# Autodesk Inventor assembly: ASY GBK 1320 long wall shield 5
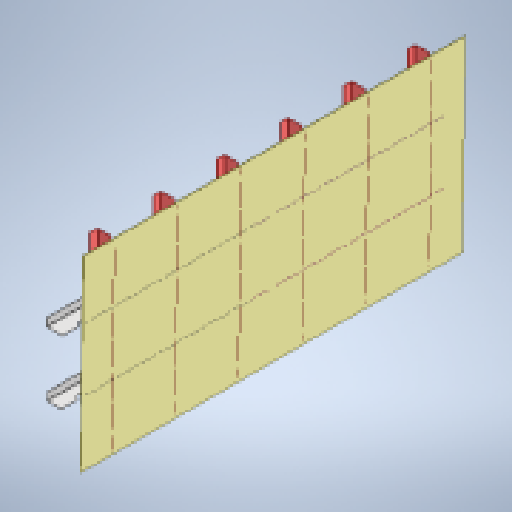
[picture p0: Inventor's stored thumbnail of the model, 512x512]
Saved by Autodesk Inventor 2026 (Build 300175000, 175)
## iProperties
Created: 2026-05-07
Part Number: ASY GBK 1320 long wall shield 5
Document SubType Name: Assembly
Designer: pokla
Mass: 215512 g
Surface Area: 139105 cm^2
Volume: 27453.8 cm^3
Density: 7.85 g/cm^3
Stock Number: 1321
Author: admin
## Documents named in this file (6)
- C:\Users\pokla\Documents\Inventor\GBK-Gubkinskiy\ASY GBK 1320 long wall shield 5.iam
- C:\Users\pokla\Documents\Inventor\GBK-Gubkinskiy\GBK 1211 shield 2.ipt
- C:\Users\pokla\Documents\Inventor\GBK-Gubkinskiy\GBK 0101 main rib.ipt
- C:\Users\pokla\Documents\Inventor\GBK-Gubkinskiy\GBK 0302 stringer 7.ipt
- C:\Users\pokla\Documents\Inventor\GBK-Gubkinskiy\GBK 0303 stringer 8.ipt
- C:\Users\pokla\Documents\Inventor\GBK-Gubkinskiy\GBK 0301 third rib.ipt
## Components (11 placed, 5 different names)
1. GBK 0302 stringer 7.ipt:1 — Жесткий:4
2. GBK 0303 stringer 8.ipt:1 — Жесткий:3
3. GBK 1211 shield 2.ipt:1 — Совмещение:1, Совмещение:2, Заподлицо:1
4. GBK 0303 stringer 8.ipt:2 — Жесткий:3
5. GBK 0302 stringer 7.ipt:2 — Жесткий:4
6. GBK 0301 third rib.ipt:1 — Совмещение:1, Совмещение:2, Заподлицо:1
7. 07.2 GBK rib:2
8. 07.2 GBK rib:3
9. 07.2 GBK rib:4
10. 07.2 GBK rib:5
11. 07.2 GBK rib:6
## Component patterns: (6 elements, first: GBK 0301 third rib.ipt:1)
## Relationships (7: WeldJoint 4, Mate 2, Flush 1)
- [WeldJoint] (4 mm): GBK 0302 stringer 7.ipt:1 ↔ GBK 0301 third rib.ipt:1
- [WeldJoint] (4 mm): GBK 0303 stringer 8.ipt:1 ↔ GBK 0301 third rib.ipt:1
- Совмещение:1 [Mate]: GBK 1211 shield 2.ipt:1 ↔ GBK 0301 third rib.ipt:1
- Совмещение:2 [Mate]: GBK 1211 shield 2.ipt:1 ↔ GBK 0301 third rib.ipt:1
- Заподлицо:1 [Flush] (254 mm): GBK 1211 shield 2.ipt:1 ↔ GBK 0301 third rib.ipt:1
- Жесткий:3 [WeldJoint]: GBK 0303 stringer 8.ipt:1 ↔ GBK 0303 stringer 8.ipt:2
- Жесткий:4 [WeldJoint]: GBK 0302 stringer 7.ipt:1 ↔ GBK 0302 stringer 7.ipt:2
## Named parameters: Шаг_шпангоутов = 496.66667 mm
